# Autodesk Inventor assembly: colsonwgeelwithhub
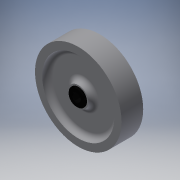
[picture p0: Inventor's stored thumbnail of the model, 180x180]
Saved by Autodesk Inventor 2019 (Build 230136000, 136)
## iProperties
Created: 2018-07-02
Part Number: colsonwgeelwithhub
Document SubType Name: Assembly
Designer: s-2512711
Author: s-2512711
## Documents named in this file (3)
- D:\Summer Drive Base V1\Summer Drivebase\colsonwgeelwithhub.iam
- D:\Summer Drive Base V1\Summer Drivebase\Colson_Live_Hub_217-3430.ipt
- D:\Summer Drive Base V1\Summer Drivebase\6inColson.ipt
## Components (2 placed, 2 different names)
1. Colson_Live_Hub_217-3430:1 — Mate:1, Mate:2, Rotation:1
2. 6inColson:1 — Mate:1, Mate:2, Rotation:1
## Relationships (3: Mate 2, RelateRotation 1)
- Mate:1: Colson_Live_Hub_217-3430:1 ↔ 6inColson:1
- Mate:2: Colson_Live_Hub_217-3430:1 ↔ 6inColson:1
- Rotation:1 [RelateRotation] (1 ul): Colson_Live_Hub_217-3430:1 ↔ 6inColson:1
